# Autodesk Inventor assembly: Assembly
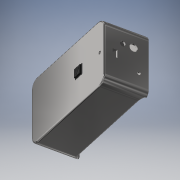
[picture p0: Inventor's stored thumbnail of the model, 180x180]
Saved by Autodesk Inventor 2019.3 (Build 233278000, 278)
## iProperties
Created: 2019-01-26
Part Number: Assembly
Document SubType Name: Assembly
Designer: Jared
Author: Jared
## iProperties of the stored document AABattery Holder.ipt
Created: 2015-01-10
Part Number: AABattery Holder
Material: Generic
Document SubType Name: Modeling
Designer: Jared
Density: 1 g/cm^3
Appearance: Default
Sending System: Kubotek KeyCreator
Preprocessor: KCM Version 1.1.1028.0
Title: X:/00DATA/CAD/Misc/AABattery Holder.stp
Author: keycreator
## Documents named in this file (22)
- **D:\Jared\Onedrive\uOttawa\GNG 2101 D\Inventor\V2\Assembly.iam*LocalDocs*xZcv0nfywGmaius0l4w4sytnpLf*AABattery Holder.ipt
- C:\Users\Jared\OneDrive\uOttawa\GNG 2101 D\Inventor\V2\Assembly.iam
- C:\Users\Jared\OneDrive\uOttawa\GNG 2101 D\Inventor\V2\Base.ipt
- C:\Users\Jared\OneDrive\uOttawa\GNG 2101 D\Inventor\V2\Carriage.ipt
- C:\Users\Jared\OneDrive\uOttawa\GNG 2101 D\Inventor\V2\Small Continuous Servo.iam
- C:\Users\Jared\OneDrive\uOttawa\GNG 2101 D\Inventor\V2\Small Continuous Servo Horn.ipt
- C:\Users\Jared\OneDrive\uOttawa\GNG 2101 D\Inventor\V2\Wire.ipt
- **C:\Users\Jared\OneDrive\uOttawa\GNG 2101 D\Inventor\V2\Assembly.iam*LocalDocs*xZcv0nfywGmaius0l4w4sytnpLf*AABattery Holder.ipt
- C:\Users\Jared\OneDrive\uOttawa\GNG 2101 D\Inventor\V2\Linear Resistor Body.ipt
- C:\Users\Jared\OneDrive\uOttawa\GNG 2101 D\Inventor\V2\Linear Resistor Post.ipt
- C:\Users\Jared\OneDrive\uOttawa\GNG 2101 D\Inventor\V2\MidPlate v2.ipt
- C:\Users\Jared\OneDrive\uOttawa\GNG 2101 D\Inventor\V2\Inner Rail 1.ipt
- C:\Users\Jared\OneDrive\uOttawa\GNG 2101 D\Inventor\V2\Inner Rails 2.ipt
- C:\Users\Jared\OneDrive\uOttawa\GNG 2101 D\Inventor\V2\Inner Rails 3.ipt
- C:\Users\Jared\OneDrive\uOttawa\GNG 2101 D\Inventor\V2\Inner Rails 4.ipt
- C:\Users\Jared\OneDrive\uOttawa\GNG 2101 D\Inventor\V2\Cover.ipt
- C:\Users\Jared\OneDrive\uOttawa\GNG 2101 D\Inventor\V2\Cover Pin.ipt
- C:\Users\Jared\OneDrive\uOttawa\GNG 2101 D\Inventor\V2\Nut.ipt
- C:\Users\Jared\OneDrive\uOttawa\GNG 2101 D\Inventor\V2\Power PCB.ipt
- C:\Users\Jared\OneDrive\uOttawa\GNG 2101 D\Inventor\V2\Main PCB.iam
- C:\Users\Jared\OneDrive\uOttawa\GNG 2101 D\Inventor\V2\Top Button.ipt
- C:\Users\Jared\OneDrive\uOttawa\GNG 2101 D\Inventor\V2\AABattery Holder.stp
## Components (24 placed, 21 different names)
1. Base:1 — Mate:18 (Moving), Mate:19, Mate:20, Mate:21, Mate:53, Mate:54, Mate:55, Mate:56, Mate:57, Mate:58, Mate:59, Mate:60, Mate:61, Mate:62, Mate:63, Mate:64, Mate:65, Mate:66, Mate:67, Mate:68, Mate:72, Mate:74, Mate:75, Mate:76, Mate:77 (Moving), Mate:78, Mate:79, Flush:18, Mate:80, Mate:81, Moving 3, Moving 2, Moving, Flush:87, Mate:85
2. Carriage:1 — Mate:7, Mate:47 (Moving), Mate:48, Mate:51, Flush:88, Mate:86
3. Small Continuous Servo:1 [sub-assembly] — Mate:5, Mate:6, Mate:18 (Moving), Mate:19, Mate:20, Flush:88, Mate:86
4. Small Continuous Servo Horn:1 — Mate:5, Mate:6, Mate:28, Flush:10
5. Wire:1 — Mate:7, Mate:28, Flush:10
6. AABattery Holder:2 — Mate:21, Mate:70, Flush:11, Flush:12
7. Linear Resistor Body:1 — Mate:44, Mate:45, Mate:46, Mate:84
8. Linear Resistor Post:1 — Mate:44, Mate:45, Mate:46, Mate:47 (Moving), Mate:48, Mate:51
9. MidPlate v2:1 — Mate:65, Mate:66, Mate:77 (Moving), Mate:84
10. Inner Rail 1:1 (Moving) — Mate:55, Mate:56, Flush:14, Moving 3
11. Inner Rails 2:1 — Mate:53, Mate:54, Mate:71, Flush:13
12. Inner Rail 1:2 (Moving) — Mate:57, Mate:58, Flush:12, Moving
13. Inner Rails 3:1 — Mate:59, Mate:60, Mate:70, Flush:11
14. Inner Rails 4:1 — Mate:61, Mate:62, Mate:73, Flush:15, Flush:16
15. Inner Rail 1:3 (Moving) — Mate:63, Mate:64, Flush:17, Moving 2
16. Cover:1 — Mate:67, Mate:68, Rotational:1, Rigid:1, Flush:83, Mate:82, Mate:83, Flush:87
17. Cover Pin:1 — Rigid:1
18. Cover Pin:2 — Rotational:1
19. AABattery Holder:4 — Mate:73, Flush:15, Flush:16, Flush:17
20. AABattery Holder:5 — Mate:71, Flush:13, Mate:72, Flush:14
21. Nut:1 — Mate:74, Mate:75, Mate:76
22. Power PCB:1 — Mate:78, Mate:79, Mate:85
23. Main PCB:1 [sub-assembly] — Flush:18, Mate:80, Mate:81
24. Top Button:1 — Flush:83, Mate:82, Mate:83
## Relationships (64: Mate 47, Flush 15, RevoluteJoint 1, WeldJoint 1)
- Mate:5: Small Continuous Servo:1 ↔ Small Continuous Servo Horn:1
- Mate:6: Small Continuous Servo:1 ↔ Small Continuous Servo Horn:1
- Mate:7: Carriage:1 ↔ Wire:1
- Mate:18 (Moving): Base:1 ↔ Small Continuous Servo:1
- Mate:19: Base:1 ↔ Small Continuous Servo:1
- Mate:20: Base:1 ↔ Small Continuous Servo:1
- Mate:21: Base:1 ↔ AABattery Holder:2
- Mate:28: Small Continuous Servo Horn:1 ↔ Wire:1
- Mate:44: Linear Resistor Body:1 ↔ Linear Resistor Post:1
- Mate:45 (0.25 mm): Linear Resistor Body:1 ↔ Linear Resistor Post:1
- Mate:46: Linear Resistor Body:1 ↔ Linear Resistor Post:1
- Mate:47 (Moving): Carriage:1 ↔ Linear Resistor Post:1
- Mate:48: Carriage:1 ↔ Linear Resistor Post:1
- Mate:51: Carriage:1 ↔ Linear Resistor Post:1
- Mate:53: Base:1 ↔ Inner Rails 2:1
- Mate:54: Base:1 ↔ Inner Rails 2:1
- Mate:55: Base:1 ↔ Inner Rail 1:1 (Moving)
- Mate:56: Base:1 ↔ Inner Rail 1:1 (Moving)
- Mate:57: Base:1 ↔ Inner Rail 1:2 (Moving)
- Mate:58: Base:1 ↔ Inner Rail 1:2 (Moving)
- Mate:59: Base:1 ↔ Inner Rails 3:1
- Mate:60: Base:1 ↔ Inner Rails 3:1
- Mate:61: Base:1 ↔ Inner Rails 4:1
- Mate:62: Base:1 ↔ Inner Rails 4:1
- Mate:63: Base:1 ↔ Inner Rail 1:3 (Moving)
- Mate:64: Base:1 ↔ Inner Rail 1:3 (Moving)
- Mate:65: Base:1 ↔ MidPlate v2:1
- Mate:66: Base:1 ↔ MidPlate v2:1
- Mate:67: Base:1 ↔ Cover:1
- Mate:68: Base:1 ↔ Cover:1
- Flush:10: Small Continuous Servo Horn:1 ↔ Wire:1
- Rotational:1 [RevoluteJoint]: Cover:1 ↔ Cover Pin:2
- Rigid:1 [WeldJoint]: Cover:1 ↔ Cover Pin:1
- Mate:70: AABattery Holder:2 ↔ Inner Rails 3:1
- Flush:11: AABattery Holder:2 ↔ Inner Rails 3:1
- Flush:12: AABattery Holder:2 ↔ Inner Rail 1:2 (Moving)
- Mate:71: Inner Rails 2:1 ↔ AABattery Holder:5
- Flush:13: Inner Rails 2:1 ↔ AABattery Holder:5
- Mate:72: Base:1 ↔ AABattery Holder:5
- Flush:14: Inner Rail 1:1 (Moving) ↔ AABattery Holder:5
- Mate:73: Inner Rails 4:1 ↔ AABattery Holder:4
- Flush:15: Inner Rails 4:1 ↔ AABattery Holder:4
- Flush:16: Inner Rails 4:1 ↔ AABattery Holder:4
- Flush:17: Inner Rail 1:3 (Moving) ↔ AABattery Holder:4
- Mate:74 (500 mm): Base:1 ↔ Nut:1
- Mate:75: Base:1 ↔ Nut:1
- Mate:76: Base:1 ↔ Nut:1
- Mate:77 (Moving) (500 mm): Base:1 ↔ MidPlate v2:1
- Mate:78: Base:1 ↔ Power PCB:1
- Mate:79: Base:1 ↔ Power PCB:1
- Flush:18 (1 mm): Base:1 ↔ Main PCB:1
- Mate:80 (500 mm): Base:1 ↔ Main PCB:1
- Mate:81 (0.5 mm): Base:1 ↔ Main PCB:1
- Flush:83: Cover:1 ↔ Top Button:1
- Mate:82: Cover:1 ↔ Top Button:1
- Mate:83: Cover:1 ↔ Top Button:1
- Moving 3 [Flush] (-500 mm): Base:1 ↔ Inner Rail 1:1 (Moving)
- Moving 2 [Flush] (-500 mm): Base:1 ↔ Inner Rail 1:3 (Moving)
- Moving [Flush] (-500 mm): Base:1 ↔ Inner Rail 1:2 (Moving)
- Mate:84: Linear Resistor Body:1 ↔ MidPlate v2:1
- Flush:87: Base:1 ↔ Cover:1
- Mate:85 (500 mm): Base:1 ↔ Power PCB:1
- Flush:88 (2.5 mm): Carriage:1 ↔ Small Continuous Servo:1
- Mate:86 (-3 mm): Carriage:1 ↔ Small Continuous Servo:1
